# Autodesk Inventor assembly: completeMoldAssembly
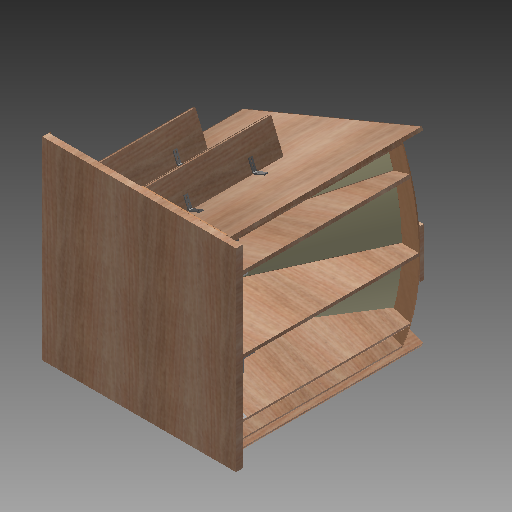
[picture p0: Inventor's stored thumbnail of the model, 512x512]
Saved by Autodesk Inventor 2019 (Build 230136000, 136)
## iProperties
Company: FABLAB Torino
Created: 2019-01-11
Part Number: completeMoldAssembly
Document SubType Name: Assembly
Designer: Giancarlo
Author: Giancarlo
Title: La Panca - Flower Vase
Subject: Construction MOld
## Documents named in this file (5)
- D:\Giancarlo Bacchio\Documenti\00 - Progetti\30-Inventor\flower vase\completeMoldAssembly.iam
- D:\Giancarlo Bacchio\Documenti\00 - Progetti\30-Inventor\flower vase\vase.ipt
- D:\Giancarlo Bacchio\Documenti\00 - Progetti\30-Inventor\flower vase\ExternalMoldAssembly.iam
- D:\Giancarlo Bacchio\Documenti\00 - Progetti\30-Inventor\flower vase\InternalBottomMoldAssembly.iam
- D:\Giancarlo Bacchio\Documenti\00 - Progetti\30-Inventor\flower vase\InternalTopMoldAssembly.iam
## Components (4 placed, 4 different names)
1. vase:1 — Mate:2, Mate:3, Mate:4, Mate:5, Mate:6, Flush:1, Mate:7, Mate:8
2. ExternalMoldAssembly:1 [sub-assembly] — Mate:2, Mate:3
3. InternalBottomMoldAssembly:1 [sub-assembly] — Mate:4, Mate:5, Mate:6
4. InternalTopMoldAssembly:1 [sub-assembly] — Flush:1, Mate:7, Mate:8
## Relationships (8: Mate 7, Flush 1)
- Mate:2: vase:1 ↔ ExternalMoldAssembly:1
- Mate:3: vase:1 ↔ ExternalMoldAssembly:1
- Mate:4: vase:1 ↔ InternalBottomMoldAssembly:1
- Mate:5: vase:1 ↔ InternalBottomMoldAssembly:1
- Mate:6: vase:1 ↔ InternalBottomMoldAssembly:1
- Flush:1: vase:1 ↔ InternalTopMoldAssembly:1
- Mate:7: vase:1 ↔ InternalTopMoldAssembly:1
- Mate:8: vase:1 ↔ InternalTopMoldAssembly:1
